# Autodesk Inventor assembly: 046-DP
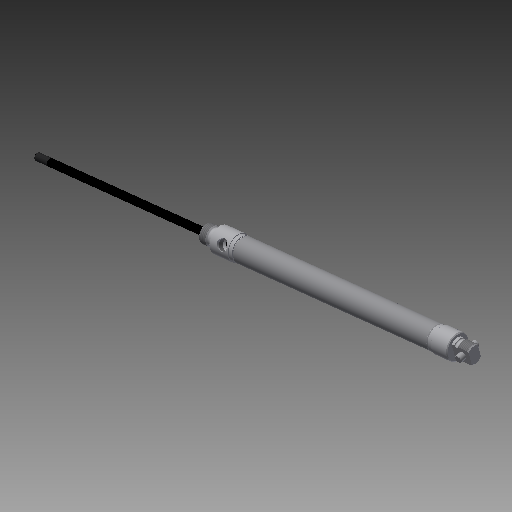
[picture p0: Inventor's stored thumbnail of the model, 512x512]
Saved by Autodesk Inventor 2017 (Build 210142000, 142)
## iProperties
Category: PARTsolutions
Company: BIMBA
Created: 2020-02-08
Part Number: 046-DP
Catalog Web Link: www.cadenas.de
Description: Original Line Standard Air Cylinders-Standard Air Cylinders
Vendor: BIMBA
Document SubType Name: Assembly
Designer: psadmin
Manufacturer: BIMBA
PSOL_IDENT_0: {$CADENAS_DATA\23d-libs\bimba\bimba_brand\bimba_imperial\bimba_full_line\original_line_cylinders\sta
PSOL_IDENT_1: ndard_air_cylinders\standard_air_cylinder_asmtab.prj},320 {VTYP=3D},{STYP=ASSTAB},{NB=046-DP},{LINA=
PSOL_IDENT_2: 046-DP},{NN=Original Line Standard Air Cylinders},{DATE=22.01.2020 09:07:35},{GEOMDATE=24.10.2019 09
PSOL_IDENT_3: :09:47},{VERSION=},{LINEID=50},{WBVAR=STROKE,ACTING,MNT,DER,NR,BM,CO,OO,VO,M,EE,EEL,K,Q,Y,G,T,HL,B,H
PSOL_IDENT_4: ,SER,SR,NT,W,STPT1,STPT2,STPT3,STPT4,MB,PB,PRC,TB,MN},{WBNUMERIC=STROKE,EEL}  {NB=046-DP},{LINA=046-
PSOL_IDENT_5: DP},{KT=DUMMY},{PN=046-DP},{PNC=046-DP},{PNA=(NO ACCESSORIES)},{DASH=-},{BORE1=0.75000000},{BORE=3/4
PSOL_IDENT_6: \" (04)},{BOREPN=04},{STROKE=6.000},{STROKEALG=[0.011:50/0.001]},{STROKE1=6.000},{ACTING=D},{ACTINGA
PSOL_IDENT_7: LG= '' , 'Single Acting' , 'R' , 'Reverse Single Acting (R)' , 'D' , 'Double Acting (D)' },{ACTINGPN=
PSOL_IDENT_8: D},{MNT=P},{MNTALG= '' , 'Front Nose Mounting' , 'P' , 'Rear Pivot Mounting (P)' , 'XP' , 'Double En
PSOL_IDENT_9: d or Pivot Mounting (XP)' , 'X' , 'Double End Mounting (X)' , 'BF' , 'Front Block Mounting (BF)' , '
PSOL_IDENT_10: BR' , 'Rear Block Mounting for Vertical Positioning (BR)' , 'BFT' , 'Front Block Trunnion Mounting (
PSOL_IDENT_11: BFT)' , 'BRT' , 'Rear Block Trunnion Mounting (BRT)' },{TYPE=},{MNTPN=P},{DER=},{DERALG= '' , 'N/A'
PSOL_IDENT_12: },{NR=},{NRALG= '' , 'N/A' },{NRPN=},{BM=},{BMALG= '' , 'N/A' },{BMPN=},{CO=},{COALG= '' , 'N/A' },{
PSOL_IDENT_13: OO=},{OOALG= '', 'N/A' },{OOPN=},{VO=Z},{VOALG= 'Z' , 'N/A' },{VOPN=},{OOVOPN=},{M=},{MALG= '', 'Wit
PSOL_IDENT_14: hout Magnet', 'M', 'With Magnet' },{EE=},{EEL=0.000},{EEMAX=44.0000},{EEALG= '', 'Without Extra Exte
PSOL_IDENT_15: nsion', 'EE', 'With Extra Extension' },{EELALG=0},{EEPN=},{EEPN1=0.000},{K=},{KALG= '', 'Standard' ,
PSOL_IDENT_16: 'K' , 'Ports Rotated 90deg K' },{KPN=},{Q=},{QALG= '' , 'N/A' },{QPN=},{Y=},{YALG= '' , 'Without Pi
PSOL_IDENT_17: vot Bushing' , 'Y' , 'With Pivot Bushing' },{YPN=},{YCON=},{F=},{FALG= '', 'Non-Coated (Standard)', '
PSOL_IDENT_18: F', 'Molycoated' },{FPN=},{G=},{GPN=},{GPN99=},{T=},{TALG= '' , 'Standard -20° to 200°F (-29° to 95°
PSOL_IDENT_19: C)' , 'N' , 'Low Temperature' , 'V' , 'High Temperature' },{NPN=},{VPN=},{HL=},{HLALG= '' , 'Without
PSOL_IDENT_20: Low Pressure Hydraulic' , 'HL' , 'With Low Pressure Hydraulic' },{B=},{BALG= '', 'W/out Bumpers' , '
PSOL_IDENT_21: B' , 'W/ Bumpers' },{BPN=},{H=},{HALG= '', 'N/A' },{HPN=},{SER=},{SERALG= '' , 'Without Spring Exten
PSOL_IDENT_22: d/Return' , 'JS' , 'With Spring Return' , 'JR' , 'With Spring Extend' },{SR=C},{SRALG= 'C' , 'Standa
PSOL_IDENT_23: rd Blackened Carbon Steel' , 'SR' , 'Stainless Steel [SR]' },{SRPN=},{SRCON=1},{NT=},{NTPN=},{W=},{W
PSOL_IDENT_24: ALG= '' , 'Without Wiper' , 'W' , 'With Wiper' },{WPN=},{E=},{EALG= '' , 'Standard Seals/Lube' , 'E'
PSOL_IDENT_25: , 'Non-Lube Seals/Lube' },{EPN=},{ST=},{STALG= '' , 'N/A' },{STPT1=},{STPT1ALG= '' , 'N/A' },{STPT2=
PSOL_IDENT_26: },{STPT2ALG= '' , 'N/A' },{STPT3=},{STPT3ALG= '' , 'N/A' },{STPT4=},{STPT4ALG= '' , 'N/A' },{STPN=},
PSOL_IDENT_27: {MB=},{MBALG= '' , 'N/A' },{MBPN=},{MBPNALL=},{MBPNALLREAR=},{PB=},{PBALG= '' , 'Without Pivot Brack
PSOL_IDENT_28: et' , 'D-167' , 'D-167' },{PBPN=},{PBPNALL=D-167},{PRC=},{PRCALG= '' , 'W/out Pivot Rod Clevis' , 'F
PSOL_IDENT_29: ,D-166-3' , 'D-166-3 (front)' },{PRCPN=},{PRCPNALL=D-166-3},{TB=},{TBALG= '' , 'N/A' },{TBPN=},{TBPN
PSOL_IDENT_30: ALL=},{MN=},{MNALG= '' , 'Without Mounting Nut' , 'F,D-9' , 'D-9 (front)' , 'R,D-9' , 'D-9 (rear)', '
PSOL_IDENT_31: 2x,D-9' , 'D-9 (front & rear)' },{MNPN=},{MNCONF=},{MNCONR=},{TLEN=7.2555},{FRAC=44.7500},{RGCON=},{
PSOL_IDENT_32: RGDACCON=R},{RHCON=P},{RHCON1=P},{RHCONON=1},{RHACCON=},{FNUTCON=0},{RNUTCON=0},{FNUTPN=D-9},{RNUTPN=
PSOL_IDENT_33: D-9},{FNUTTRANS=0.0000},{RNUTTRANS=0.0000},{VHOLECON=0},{A1=1.5940},{A1N=0.8750},{A1P=1.5940},{A1B=1
PSOL_IDENT_34: .5940},{A4=0.2525},{A4N=0.3130},{A4P=0.2525},{A5=0.0300},{A1H=1.594},{A1NH=0.5310},{A1PH=1.5940},{A1
PSOL_IDENT_35: BH=1.0940},{A1SH=1.2190},{A2H=0.2190},{A2NH=0.2190},{LENGTH=3.7500},{LENGTH1=3.7500},{LENGTH2=3.8100
PSOL_IDENT_36: },{MUL=6.0000},{MUL11=6.0000},{MUL22=16.14},{MUL33=10.1400},{MUL2=6.0000},{MUL211=6.0000},{MUL222=2.
PSOL_IDENT_37: 6900},{MUL233=1.6900},{SSS=12.0000},{RGLEN=1.3715},{RHLEN=1.1230},{SSS1=7.0000},{A13=1.3120},{DIF=0.
PSOL_IDENT_38: 0000},{G5=0.6250},{ON=0},{SSADD=0.0000},{BADD=0.0000},{MADD=0.0000},{NVADD=0.0000},{TRACKL=6.9655},{
PSOL_IDENT_39: TRACKCON=D-74168},{TRIMCON=0},{TRIMCON1=0},{PINCON=D-51},{FSPACE=0.6305},{SPACE=0.1071},{TEXT=0.1875
PSOL_IDENT_40: },{S1=1.0000},{D1=0.8325},{D1N=0.8050},{D1B=0.8625},{D1P=0.8325},{FA=0.940},{RA=0.9400},{PPATH=stand
PSOL_IDENT_41: ard_air_cylinder_asmtpl.prj},{MATALGHTML=<b>Standard Original Line:</b><dl><dt>Rod:</dt><dd>- Stainl
PSOL_IDENT_42: ess Steel</dd><dd>&nbsp;&nbsp;(5/16 9/16 Bores)</dd><dd>- High Strength Carbon Steel</dd><dd>&nbsp;&
PSOL_IDENT_43: nbsp;(3/4 3 Bore)</dd><dd>- Stainless Steel</dd><dd>&nbsp;&nbsp;(X style DXP/DX/DXDE)</dd><dt>Bearin
PSOL_IDENT_44: gs:</dt><dd>- Sintered Bronze</dd><dt>Body:</dt><dd>- 304 Stainless Steel</dd><dt>End Caps:</dt><dd>
PSOL_IDENT_45: - Aluminum</dd><dt>Seals:</dt><dd>- Buna N</dd></dl>},{ASSCFGPRA=04DP},{MBPNA=},{MNPNA=},{PRCPNA=},{
PSOL_IDENT_46: ASSOPTACC=STPT4},{A=9.75},{HADD=0.0000},{WFL=0.25},{QADD=0.000},{QADD1=0.440},{TEST=6.0000},{MNTB=},
PSOL_IDENT_47: {STDNUTF=0},{STDNUTR=0},{STRK2D=0},{X2D=2},{STROKESW=6.000},{EESW=0.000},{FCD=0},{BCD=0},{RCD=0},{CU
PSOL_IDENT_48: STADD=5.000},{FT=1/4-28 UNF-2A},{FT1=1/4-28 UNF-2A},{FT2=5/8-18 UNF-2A},{PORT=1/8 NPT},{FT11=1/2-20
PSOL_IDENT_49: UNF-2A},{FT12=5/8-18 UNF-2A},{B1=}
NN: Original Line Standard Air Cylinders
NT: Threaded (Standard)
NB: 046-DP
NBSYN: $PNC.
LINA: 046-DP
PN: 046-DP
PNA: (NO ACCESSORIES)
BORE: 3/4" (04)
STROKE: 6
ACTING: Double Acting (D)
MNT: Rear Pivot Mounting (P)
DER: N/A
NR: N/A
BM: N/A
CO: N/A
OO: N/A
VO: N/A
M: Without Magnet
EE: Without Extra Extension
EEL: 0
K: Standard
Q: N/A
Y: Without Pivot Bushing
G: Standard Lube
T: Standard -20° to 200°F (-29° to 95°C)
HL: Without Low Pressure Hydraulic
B: W/out Bumpers
H: N/A
SER: Without Spring Extend/Return
SR: Standard Blackened Carbon Steel
W: Without Wiper
STPT1: N/A
STPT2: N/A
STPT3: N/A
STPT4: N/A
MB: N/A
PB: Without Pivot Bracket
PRC: W/out Pivot Rod Clevis
TB: N/A
MN: Without Mounting Nut
A: 9.75
SUPPLIER: BIMBA
ARTICLENO: 046-DP
BOMINFO: 046-DP
CREATOR: CADENAS GmbH
Title: 046-DP
Author: Cadenas PARTsolutions
Comments: Standard Air Cylinders
## Documents named in this file (7)
- \\ad.ocdsb.ca\studenthome\3\S338674153\FRC 2020\FullRobotRefactor\Control Panel Revision\046-DP.iam
- \\ad.ocdsb.ca\studenthome\3\S338674153\FRC 2020\FullRobotRefactor\Control Panel Revision\046-DPC0000000_0_dummy.ipt
- \\ad.ocdsb.ca\studenthome\3\S338674153\FRC 2020\FullRobotRefactor\Control Panel Revision\04R000-0_rod_guide.ipt
- \\ad.ocdsb.ca\studenthome\3\S338674153\FRC 2020\FullRobotRefactor\Control Panel Revision\04R-7_25550C.ipt
- \\ad.ocdsb.ca\studenthome\3\S338674153\FRC 2020\FullRobotRefactor\Control Panel Revision\04P0000_rear_head.ipt
- \\ad.ocdsb.ca\studenthome\3\S338674153\FRC 2020\FullRobotRefactor\Control Panel Revision\D-51.ipt
- \\ad.ocdsb.ca\studenthome\3\S338674153\FRC 2020\FullRobotRefactor\Control Panel Revision\C-046-DP0000_rod.ipt
## Components (6 placed, 6 different names)
1. 046-DPC0000000_0_dummy:1
2. 04R000-0_rod_guide:1 — Mate:4, Mate:5, Mate:7
3. 04R-7_25550C:1 — Mate:1, Mate:2, Mate:4, Mate:6, Mate:7
4. 04P0000_rear_head:1 — Mate:1, Mate:2, Mate:3, Mate:8
5. D-51:1 — Mate:3, Mate:8
6. C-046-DP0000_rod:1 — Mate:5, Mate:6
## Relationships (8: Mate 8)
- Mate:1: 04R-7_25550C:1 ↔ 04P0000_rear_head:1
- Mate:2: 04R-7_25550C:1 ↔ 04P0000_rear_head:1
- Mate:3: 04P0000_rear_head:1 ↔ D-51:1
- Mate:4: 04R000-0_rod_guide:1 ↔ 04R-7_25550C:1
- Mate:5: 04R000-0_rod_guide:1 ↔ C-046-DP0000_rod:1
- Mate:6 (127 mm): 04R-7_25550C:1 ↔ C-046-DP0000_rod:1
- Mate:7: 04R000-0_rod_guide:1 ↔ 04R-7_25550C:1
- Mate:8 (-14.3129 mm): 04P0000_rear_head:1 ↔ D-51:1
